# Autodesk Inventor assembly: 18650ASSEMBLYfordrawing
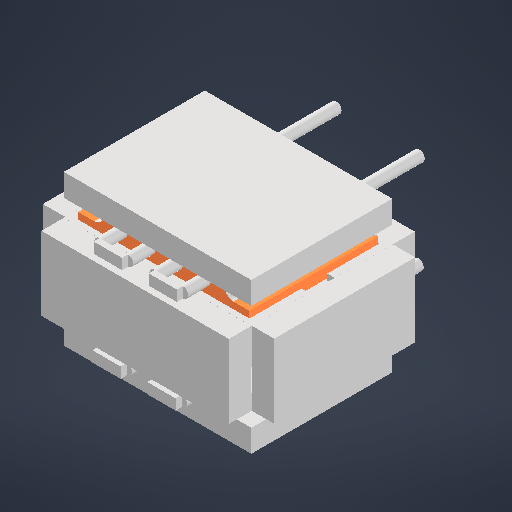
[picture p0: Inventor's stored thumbnail of the model, 512x512]
Saved by Autodesk Inventor 2025.2 (Build 292293000, 293)
## iProperties
Created: 2025-03-05
Part Number: 18650ASSEMBLYfordrawing
Document SubType Name: Assembly
Designer: cbast
Author: cbast
## Documents named in this file (10)
- C:\Users\cbast\OneDrive\Documents\GitHub\Smart-Pack-for-Advanced-Research-and-Control\variations\Camden\V0.2\18650ASSEMBLYfordrawing.iam
- C:\Users\cbast\OneDrive\Documents\GitHub\Smart-Pack-for-Advanced-Research-and-Control\variations\Camden\V0.2\PILLARSCELLCASE18650.ipt
- C:\Users\cbast\OneDrive\Documents\GitHub\Smart-Pack-for-Advanced-Research-and-Control\variations\Camden\V0.1\18650(PINK).ipt
- C:\Users\cbast\OneDrive\Documents\GitHub\Smart-Pack-for-Advanced-Research-and-Control\variations\Camden\V0.1\343thermalpad.ipt
- C:\Users\cbast\OneDrive\Documents\GitHub\Smart-Pack-for-Advanced-Research-and-Control\variations\Camden\V0.1\cooling plate.ipt
- C:\Users\cbast\OneDrive\Documents\GitHub\Smart-Pack-for-Advanced-Research-and-Control\variations\Camden\V0.2\insulation.ipt
- C:\Users\cbast\OneDrive\Documents\GitHub\Smart-Pack-for-Advanced-Research-and-Control\variations\Camden\V0.2\insulation2.ipt
- C:\Users\cbast\OneDrive\Documents\GitHub\Smart-Pack-for-Advanced-Research-and-Control\variations\Camden\V0.2\Part3.ipt
- C:\Users\cbast\OneDrive\Documents\GitHub\Smart-Pack-for-Advanced-Research-and-Control\variations\Camden\V0.2\Part4.ipt
- C:\Users\cbast\OneDrive\Documents\GitHub\Smart-Pack-for-Advanced-Research-and-Control\variations\Camden\V0.2\Part5.ipt
## Components (22 placed, 9 different names)
1. PILLARSCELLCASE18650:1 — Mate:1, Mate:2, Mate:3, Mate:4, Mate:5, Mate:6, Mate:7, Mate:8, Mate:9, Mate:10, Mate:12, Mate:13, Mate:26, Mate:27, Mate:30, Mate:31, Flush:3, Flush:4
2. PILLARSCELLCASE18650:2 — Mate:11, Mate:12, Mate:13, Mate:14, Mate:15, Mate:16, Mate:17, Mate:18, Mate:19, Mate:20, Mate:21, Mate:22, Mate:23, Mate:28, Mate:29
3. 18650(PINK):1 — Mate:9, Mate:17
4. 18650(PINK):2 — Mate:3, Mate:19
5. 18650(PINK):3 — Mate:10, Mate:14
6. 18650(PINK):4 — Mate:2, Mate:22
7. 18650(PINK):5 — Mate:8, Mate:16
8. 18650(PINK):6 — Mate:1, Mate:20
9. 18650(PINK):7 — Mate:7, Mate:18, Mate:25
10. 18650(PINK):8 — Mate:6, Mate:21, Mate:24
11. 18650(PINK):9 — Mate:5, Mate:11, Mate:23
12. 18650(PINK):10 — Mate:4, Mate:15
13. 343thermalpad:1 — Mate:24
14. 343thermalpad:2 — Mate:25
15. cooling plate:1 — Mate:26, Mate:27, Flush:1
16. cooling plate:2 — Mate:28, Mate:29, Flush:2
17. insulation:1 — Mate:30
18. insulation:2 — Mate:31
19. insulation2:1 — Flush:1
20. Part3:1 — Flush:2
21. Part4:1 — Flush:3
22. Part5:1 — Flush:4
## Relationships (35: Mate 31, Flush 4)
- Mate:1: PILLARSCELLCASE18650:1 ↔ 18650(PINK):6
- Mate:2: PILLARSCELLCASE18650:1 ↔ 18650(PINK):4
- Mate:3: PILLARSCELLCASE18650:1 ↔ 18650(PINK):2
- Mate:4: PILLARSCELLCASE18650:1 ↔ 18650(PINK):10
- Mate:5: PILLARSCELLCASE18650:1 ↔ 18650(PINK):9
- Mate:6: PILLARSCELLCASE18650:1 ↔ 18650(PINK):8
- Mate:7: PILLARSCELLCASE18650:1 ↔ 18650(PINK):7
- Mate:8: PILLARSCELLCASE18650:1 ↔ 18650(PINK):5
- Mate:9: PILLARSCELLCASE18650:1 ↔ 18650(PINK):1
- Mate:10: PILLARSCELLCASE18650:1 ↔ 18650(PINK):3
- Mate:11: PILLARSCELLCASE18650:2 ↔ 18650(PINK):9
- Mate:12: PILLARSCELLCASE18650:1 ↔ PILLARSCELLCASE18650:2
- Mate:13: PILLARSCELLCASE18650:1 ↔ PILLARSCELLCASE18650:2
- Mate:14 (5.75 mm): PILLARSCELLCASE18650:2 ↔ 18650(PINK):3
- Mate:15 (5.75 mm): PILLARSCELLCASE18650:2 ↔ 18650(PINK):10
- Mate:16 (5.75 mm): PILLARSCELLCASE18650:2 ↔ 18650(PINK):5
- Mate:17 (5.75 mm): PILLARSCELLCASE18650:2 ↔ 18650(PINK):1
- Mate:18 (5.75 mm): PILLARSCELLCASE18650:2 ↔ 18650(PINK):7
- Mate:19 (5.75 mm): PILLARSCELLCASE18650:2 ↔ 18650(PINK):2
- Mate:20 (5.75 mm): PILLARSCELLCASE18650:2 ↔ 18650(PINK):6
- Mate:21 (5.75 mm): PILLARSCELLCASE18650:2 ↔ 18650(PINK):8
- Mate:22 (5.75 mm): PILLARSCELLCASE18650:2 ↔ 18650(PINK):4
- Mate:23 (5.75 mm): PILLARSCELLCASE18650:2 ↔ 18650(PINK):9
- Mate:24: 18650(PINK):8 ↔ 343thermalpad:1
- Mate:25: 18650(PINK):7 ↔ 343thermalpad:2
- Mate:26: PILLARSCELLCASE18650:1 ↔ cooling plate:1
- Mate:27: PILLARSCELLCASE18650:1 ↔ cooling plate:1
- Mate:28: PILLARSCELLCASE18650:2 ↔ cooling plate:2
- Mate:29: PILLARSCELLCASE18650:2 ↔ cooling plate:2
- Mate:30: PILLARSCELLCASE18650:1 ↔ insulation:1
- Mate:31: PILLARSCELLCASE18650:1 ↔ insulation:2
- Flush:1: cooling plate:1 ↔ insulation2:1
- Flush:2: cooling plate:2 ↔ Part3:1
- Flush:3: PILLARSCELLCASE18650:1 ↔ Part4:1
- Flush:4: PILLARSCELLCASE18650:1 ↔ Part5:1
